# Autodesk Inventor assembly: hub_shaft_assy
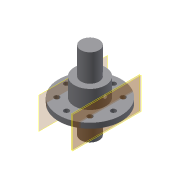
[picture p0: Inventor's stored thumbnail of the model, 180x180]
Saved by Autodesk Inventor 2022 (Build 260148000, 148)
## iProperties
Created: 2005-10-24
Part Number: hub_shaft_assy
Document SubType Name: Assembly
Designer: dchu
Author: dchu
## Documents named in this file (3)
- C:\Autodesk Inventor 2022 Advanced Assembly Modeling Practice Files\hub_shaft_assy.iam
- C:\Autodesk Inventor 2022 Advanced Assembly Modeling Practice Files\hub.ipt
- C:\Autodesk Inventor 2022 Advanced Assembly Modeling Practice Files\shaft.ipt
## Components (2 placed, 2 different names)
1. hub:1 — Mate:1, Tangent:1, Tangent:2
2. shaft:1 — Mate:1, Tangent:1
## Relationships (6: Tangent 2, Flush 2, Mate 1, Angle 1)
- Mate:1: hub:1 ↔ shaft:1
- Tangent:1: hub:1 ↔ shaft:1
- Angle:1 (0 deg)
- Tangent:2: hub:1
- Flush:1 (2.5 mm)
- Flush:2 (-65 mm)
